# Autodesk Inventor assembly: ASY MSC 010 cone
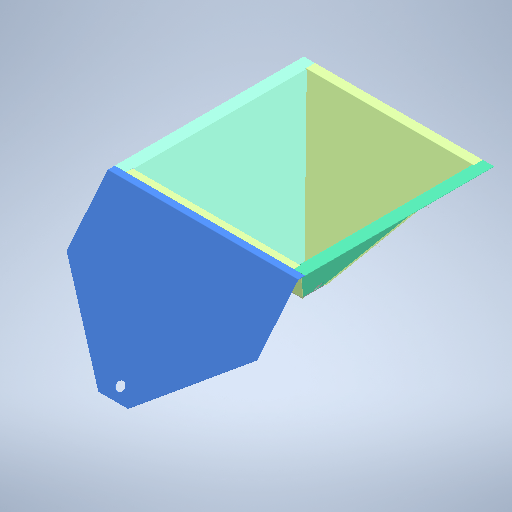
[picture p0: Inventor's stored thumbnail of the model, 512x512]
Saved by Autodesk Inventor 2025 (Build 290162010, 162A)
## iProperties
Created: 2024-05-19
Part Number: ASY MSC 010 cone
Document SubType Name: Assembly
Designer: admin
Mass: 24706.5 g
Surface Area: 124528 cm^2
Volume: 24706.5 cm^3
Density: 1 g/cm^3
Stock Number: ASY МОО 010 конус
Author: admin
## Documents named in this file (14)
- C:\Users\admin\YandexDisk-badmisterfox\домашниий пк\Inventor\Manturovo\Manturovo_Se-clar\ASY MSC 010 cone.iam
- C:\Users\admin\YandexDisk-badmisterfox\домашниий пк\Inventor\Manturovo\Manturovo_Se-clar\конус\MSC 014 cone IN right board.ipt
- C:\Users\admin\YandexDisk-badmisterfox\домашниий пк\Inventor\Manturovo\Manturovo_Se-clar\конус\MSC 011 cone IN bottom.ipt
- C:\Users\admin\YandexDisk-badmisterfox\домашниий пк\Inventor\Manturovo\Manturovo_Se-clar\конус\MSC 013 cone IN left board.ipt
- C:\Users\admin\YandexDisk-badmisterfox\домашниий пк\Inventor\Manturovo\Manturovo_Se-clar\конус\MSC 012 cone IN back.ipt
- C:\Users\admin\YandexDisk-badmisterfox\домашниий пк\Inventor\Manturovo\Manturovo_Se-clar\конус\MSC 019 cone sketch.ipt
- C:\Users\admin\YandexDisk-badmisterfox\домашниий пк\Inventor\Manturovo\Manturovo_Se-clar\конус\MSC 015 cone IN bow.ipt
- C:\Users\admin\YandexDisk-badmisterfox\домашниий пк\Inventor\Manturovo\Manturovo_Se-clar\конус\MSC 016 cone exit back.ipt
- C:\Users\admin\YandexDisk-badmisterfox\домашниий пк\Inventor\Manturovo\Manturovo_Se-clar\DXF файлы\MSC 0691 stringer cone.ipt
- C:\Users\admin\YandexDisk-badmisterfox\домашниий пк\Inventor\Manturovo\Manturovo_Se-clar\DXF файлы\MSC 0561 rib cone.ipt
- C:\Users\admin\YandexDisk-badmisterfox\домашниий пк\Inventor\Manturovo\Manturovo_Se-clar\DXF файлы\MSC 0692 stringer cone.ipt
- C:\Users\admin\YandexDisk-badmisterfox\домашниий пк\Inventor\Manturovo\Manturovo_Se-clar\DXF файлы\MSC 0562 rib cone.ipt
- C:\Users\admin\YandexDisk-badmisterfox\домашниий пк\Inventor\Manturovo\Manturovo_Se-clar\DXF файлы\MSC 0563 rib cone.ipt
- C:\Users\admin\YandexDisk-badmisterfox\домашниий пк\Inventor\Manturovo\Manturovo_Se-clar\DXF файлы\MSC 0564 rib cone.ipt
## Components (15 placed, 13 different names)
1. MSC 019 cone sketch.ipt:1 — Flush:8, Flush:9, Mate:1
2. MSC 012 cone IN back.ipt:1 — Flush:6, Flush:10, Mate:2, Flush:12, Mate:23, Mate:26
3. MSC 011 cone IN bottom.ipt:1 — Flush:4, Flush:5, Flush:11
4. MSC 014 cone IN right board.ipt:1 — Flush:12, Flush:13, Flush:15, Mate:24
5. MSC 013 cone IN left board.ipt:1 — Mate:4, Flush:14, Mate:5
6. MSC 015 cone IN bow.ipt:1 — Mate:3, Mate:6, Flush:16, Flush:17, Rigid:1
7. MSC 016 cone exit back.ipt:1 — Rigid:1
8. MSC 0562 rib cone:1
9. MSC 0561 rib cone:1
10. MSC 0691 stringer cone:1 — Mate:23, Rigid:2, Mate:25, Mate:26
11. MSC 0564 rib cone:1
12. MSC 0563 rib cone:1
13. MSC 0692 stringer cone:1
14. MSC 0691 stringer cone:2 — Mate:24, Mate:25
15. MSC 0691 stringer cone:3 — Rigid:2
## Relationships (38: Mate 21, Flush 15, WeldJoint 2)
- Flush:4: MSC 011 cone IN bottom.ipt:1
- Flush:5: MSC 011 cone IN bottom.ipt:1
- Flush:6: MSC 012 cone IN back.ipt:1
- Flush:8: MSC 019 cone sketch.ipt:1
- Flush:9: MSC 019 cone sketch.ipt:1
- Mate:1: MSC 019 cone sketch.ipt:1
- Flush:10: MSC 012 cone IN back.ipt:1
- Mate:2: MSC 012 cone IN back.ipt:1
- Flush:11 (-230 mm): MSC 011 cone IN bottom.ipt:1
- Mate:3: MSC 015 cone IN bow.ipt:1
- Flush:12: MSC 012 cone IN back.ipt:1 ↔ MSC 014 cone IN right board.ipt:1
- Flush:13: MSC 014 cone IN right board.ipt:1
- Mate:4: MSC 013 cone IN left board.ipt:1
- Flush:14: MSC 013 cone IN left board.ipt:1
- Mate:5: MSC 013 cone IN left board.ipt:1
- Flush:15: MSC 014 cone IN right board.ipt:1
- Mate:6: MSC 015 cone IN bow.ipt:1
- Flush:16: MSC 015 cone IN bow.ipt:1
- Flush:17: MSC 015 cone IN bow.ipt:1
- Rigid:1 [WeldJoint]: MSC 015 cone IN bow.ipt:1 ↔ MSC 016 cone exit back.ipt:1
- [Mate]: MSC 012 cone IN back.ipt:1 ↔ MSC 0561 rib cone:1
- [Mate]: MSC 0561 rib cone:1
- [Mate]: MSC 012 cone IN back.ipt:1 ↔ MSC 0562 rib cone:1
- [Mate]: MSC 0562 rib cone:1
- [Mate]: MSC 014 cone IN right board.ipt:1 ↔ MSC 0692 stringer cone:1
- [Mate]: MSC 0692 stringer cone:1
- [Mate]: MSC 014 cone IN right board.ipt:1 ↔ MSC 0692 stringer cone:1
- [Mate]: MSC 014 cone IN right board.ipt:1 ↔ MSC 0563 rib cone:1
- [Mate] (752.254 mm): MSC 014 cone IN right board.ipt:1 ↔ MSC 0563 rib cone:1
- [Flush]: MSC 014 cone IN right board.ipt:1 ↔ MSC 0563 rib cone:1
- [Mate]: MSC 014 cone IN right board.ipt:1 ↔ MSC 0564 rib cone:1
- [Mate] (372.254 mm): MSC 014 cone IN right board.ipt:1 ↔ MSC 0564 rib cone:1
- [Flush]: MSC 014 cone IN right board.ipt:1 ↔ MSC 0564 rib cone:1
- Mate:23: MSC 012 cone IN back.ipt:1 ↔ MSC 0691 stringer cone:1
- Mate:24: MSC 014 cone IN right board.ipt:1 ↔ MSC 0691 stringer cone:2
- Rigid:2 [WeldJoint] (380 mm): MSC 0691 stringer cone:1 ↔ MSC 0691 stringer cone:3
- Mate:25: MSC 0691 stringer cone:1 ↔ MSC 0691 stringer cone:2
- Mate:26 (20 mm): MSC 012 cone IN back.ipt:1 ↔ MSC 0691 stringer cone:1
